# Autodesk Inventor assembly: Joining Plate for 4040 Assembly - B
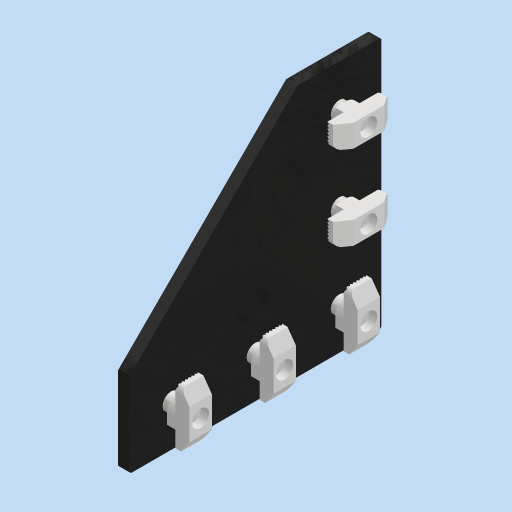
[picture p0: Inventor's stored thumbnail of the model, 512x512]
Saved by Autodesk Inventor 2023.2 (Build 272271000, 271)
## iProperties
Created: 2023-11-20
Part Number: Joining Plate for 4040 Assembly - B
Document SubType Name: Assembly
Designer: Nils Bade
Author: Nils Bade
## Documents named in this file (4)
- C:\Users\nilsb\Documents\Inventor\Projektarbeit-Bade\RatRig_modified\Joining Plate for 4040 Assembly - B_mir.iam
- C:\Users\nilsb\Documents\Inventor\Projektarbeit-Bade\RatRig_Standards\Joining Plate for 3030 - 90 Degree - Black Anodized v2.ipt
- C:\Users\nilsb\Documents\Inventor\Projektarbeit-Bade\Schrauben\Cap Head Screw M6x12 v2.ipt
- C:\Users\nilsb\Documents\Inventor\Projektarbeit-Bade\RatRig_modified\T-NUT - DropIn 4040 SERIES - M6.ipt
## Components (11 placed, 3 different names)
1. Joining Plate for 3030 - 90 Degree - Black Anodized v2:2 — Passend:21, Passend:22, Passend:23, Passend:24, Passend:25, Passend:26, Passend:27, Passend:28, Passend:29, Passend:30, Passend:31, Passend:32, Passend:35, Passend:36, Passend:37
2. Cap Head Screw M6x12 v2:1 — Passend:21, Passend:26, Passend:34
3. Cap Head Screw M6x12 v2:2 — Passend:22, Passend:30, Passend:39
4. Cap Head Screw M6x12 v2:3 — Passend:24, Passend:28, Passend:38
5. Cap Head Screw M6x12 v2:4 — Passend:23, Passend:29, Passend:40
6. Cap Head Screw M6x12 v2:5 — Passend:25, Passend:27, Passend:33
7. T-NUT - DROP IN TYPE FOR 40 SERIES - M6:1 — Passend:31, Passend:34, Winkel:5
8. T-NUT - DROP IN TYPE FOR 40 SERIES - M6:2 — Passend:32, Passend:33, Winkel:4
9. T-NUT - DROP IN TYPE FOR 40 SERIES - M6:3 — Passend:37, Passend:38, Winkel:3
10. T-NUT - DROP IN TYPE FOR 40 SERIES - M6:4 — Passend:36, Passend:40, Winkel:2
11. T-NUT - DROP IN TYPE FOR 40 SERIES - M6:5 — Passend:35, Passend:39, Winkel:1
## Relationships (25: Mate 20, Angle 5)
- Passend:21 [Mate]: Joining Plate for 3030 - 90 Degree - Black Anodized v2:2 ↔ Cap Head Screw M6x12 v2:1
- Passend:22 [Mate]: Joining Plate for 3030 - 90 Degree - Black Anodized v2:2 ↔ Cap Head Screw M6x12 v2:2
- Passend:23 [Mate]: Joining Plate for 3030 - 90 Degree - Black Anodized v2:2 ↔ Cap Head Screw M6x12 v2:4
- Passend:24 [Mate]: Joining Plate for 3030 - 90 Degree - Black Anodized v2:2 ↔ Cap Head Screw M6x12 v2:3
- Passend:25 [Mate]: Joining Plate for 3030 - 90 Degree - Black Anodized v2:2 ↔ Cap Head Screw M6x12 v2:5
- Passend:26 [Mate]: Joining Plate for 3030 - 90 Degree - Black Anodized v2:2 ↔ Cap Head Screw M6x12 v2:1
- Passend:27 [Mate]: Joining Plate for 3030 - 90 Degree - Black Anodized v2:2 ↔ Cap Head Screw M6x12 v2:5
- Passend:28 [Mate]: Joining Plate for 3030 - 90 Degree - Black Anodized v2:2 ↔ Cap Head Screw M6x12 v2:3
- Passend:29 [Mate]: Joining Plate for 3030 - 90 Degree - Black Anodized v2:2 ↔ Cap Head Screw M6x12 v2:4
- Passend:30 [Mate]: Joining Plate for 3030 - 90 Degree - Black Anodized v2:2 ↔ Cap Head Screw M6x12 v2:2
- Passend:31 [Mate] (5.5 mm): Joining Plate for 3030 - 90 Degree - Black Anodized v2:2 ↔ T-NUT - DROP IN TYPE FOR 40 SERIES - M6:1
- Passend:32 [Mate] (5.5 mm): Joining Plate for 3030 - 90 Degree - Black Anodized v2:2 ↔ T-NUT - DROP IN TYPE FOR 40 SERIES - M6:2
- Passend:33 [Mate]: Cap Head Screw M6x12 v2:5 ↔ T-NUT - DROP IN TYPE FOR 40 SERIES - M6:2
- Passend:34 [Mate]: Cap Head Screw M6x12 v2:1 ↔ T-NUT - DROP IN TYPE FOR 40 SERIES - M6:1
- Passend:35 [Mate] (5.5 mm): Joining Plate for 3030 - 90 Degree - Black Anodized v2:2 ↔ T-NUT - DROP IN TYPE FOR 40 SERIES - M6:5
- Passend:36 [Mate] (5.5 mm): Joining Plate for 3030 - 90 Degree - Black Anodized v2:2 ↔ T-NUT - DROP IN TYPE FOR 40 SERIES - M6:4
- Passend:37 [Mate] (5.5 mm): Joining Plate for 3030 - 90 Degree - Black Anodized v2:2 ↔ T-NUT - DROP IN TYPE FOR 40 SERIES - M6:3
- Passend:38 [Mate]: Cap Head Screw M6x12 v2:3 ↔ T-NUT - DROP IN TYPE FOR 40 SERIES - M6:3
- Passend:39 [Mate]: Cap Head Screw M6x12 v2:2 ↔ T-NUT - DROP IN TYPE FOR 40 SERIES - M6:5
- Passend:40 [Mate]: Cap Head Screw M6x12 v2:4 ↔ T-NUT - DROP IN TYPE FOR 40 SERIES - M6:4
- Winkel:1 [Angle] (0 deg): T-NUT - DROP IN TYPE FOR 40 SERIES - M6:5
- Winkel:2 [Angle] (0 deg): T-NUT - DROP IN TYPE FOR 40 SERIES - M6:4
- Winkel:3 [Angle] (0 deg): T-NUT - DROP IN TYPE FOR 40 SERIES - M6:3
- Winkel:4 [Angle] (0 deg): T-NUT - DROP IN TYPE FOR 40 SERIES - M6:2
- Winkel:5 [Angle] (0 deg): T-NUT - DROP IN TYPE FOR 40 SERIES - M6:1
